# Autodesk Inventor assembly: Montagem eletrolisador sem membrana - sem base
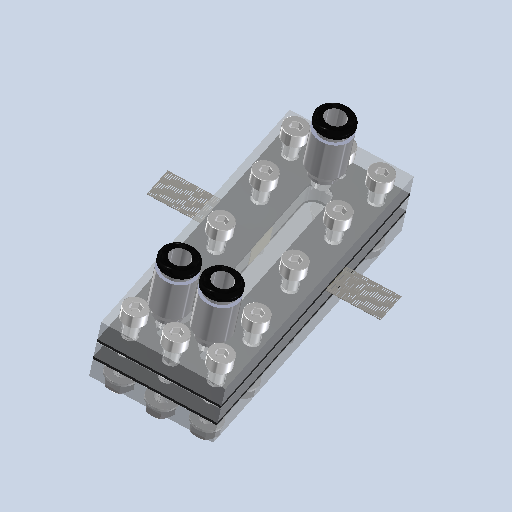
[picture p0: Inventor's stored thumbnail of the model, 512x512]
Saved by Autodesk Inventor 2025 (Build 290162010, 162A)
## iProperties
Created: 2024-12-11
Part Number: Montagem eletrolisador sem membrana - sem base
Document SubType Name: Assembly
Designer: November
Author: November
## Documents named in this file (10)
- G:\Meu Drive\1_Tese 2024\CAD - Eletrolisador\Montagem eletrolisador sem membrana - sem base.iam
- G:\Meu Drive\1_Tese 2024\CAD - Eletrolisador\borracha vedação.ipt
- G:\Meu Drive\1_Tese 2024\CAD - Eletrolisador\acrilico canal.ipt
- G:\Meu Drive\1_Tese 2024\CAD - Eletrolisador\eletrodo - nickel e titanio.ipt
- G:\Meu Drive\1_Tese 2024\CAD - Eletrolisador\acrilico frontal.ipt
- G:\Meu Drive\1_Tese 2024\CAD - Eletrolisador\Screw_DIN_912_M4x25_A2\Screw_DIN_912_M4x25_A2.ipt
- G:\Meu Drive\1_Tese 2024\CAD - Eletrolisador\Engate rápido M5\Engate rápido M5.ipt
- G:\Meu Drive\1_Tese 2024\CAD - Eletrolisador\Arruela m4.ipt
- G:\Meu Drive\1_Tese 2024\CAD - Eletrolisador\PORCA SEXTAVADA M4\PORCA SEXTAVADA M4.ipt
- G:\Meu Drive\1_Tese 2024\CAD - Eletrolisador\acrilico base.ipt
## Components (46 placed, 9 different names)
1. borracha vedação:1 — Alinhado:3, Alinhado:4, Coincidente:6, Coincidente:60
2. acrilico canal:1 — Alinhado:3, Alinhado:4, Coincidente:2, Coincidente:3, Alinhado:5, Coincidente:4, Coincidente:5, Coincidente:6, Alinhado:6, Alinhado:7, Coincidente:61, Coincidente:62
3. eletrodo - nickel e titanio:1 — Coincidente:2, Coincidente:3, Alinhado:5, Coincidente:7
4. eletrodo - nickel e titanio:2 — Coincidente:4, Coincidente:5, Coincidente:7, Coincidente:8
5. borracha vedação:2 — Coincidente:8, Alinhado:6, Alinhado:7, Coincidente:9, Alinhado:8, Alinhado:9, Coincidente:62
6. acrilico frontal:1 — Coincidente:9, Alinhado:8, Alinhado:9, Coincidente:10, Coincidente:11, Coincidente:12, Coincidente:13, Coincidente:14, Coincidente:15, Coincidente:16, Coincidente:17, Coincidente:18, Coincidente:19, Coincidente:20, Coincidente:21, Coincidente:22, Coincidente:23, Coincidente:24, Coincidente:25, Coincidente:26
7. Screw_DIN_912_M4x25_A2:1 — Coincidente:10, Coincidente:11, Alinhado:10, Alinhado:12, Coincidente:27, Coincidente:40
8. Screw_DIN_912_M4x25_A2:2 — Coincidente:12, Alinhado:10, Alinhado:11, Coincidente:38, Coincidente:41
9. Screw_DIN_912_M4x25_A2:3 — Coincidente:13, Alinhado:11, Coincidente:37, Coincidente:42
10. Screw_DIN_912_M4x25_A2:4 — Coincidente:14, Alinhado:13, Coincidente:36, Coincidente:59
11. Screw_DIN_912_M4x25_A2:5 — Coincidente:15, Alinhado:14, Alinhado:20, Coincidente:35, Coincidente:51
12. Screw_DIN_912_M4x25_A2:6 — Coincidente:16, Alinhado:16, Alinhado:20, Coincidente:34, Coincidente:50
13. Screw_DIN_912_M4x25_A2:7 — Coincidente:17, Alinhado:16, Alinhado:17, Coincidente:33, Coincidente:49
14. Screw_DIN_912_M4x25_A2:8 — Coincidente:18, Alinhado:17, Alinhado:18, Coincidente:32, Coincidente:48
15. Screw_DIN_912_M4x25_A2:9 — Coincidente:19, Alinhado:18, Alinhado:19, Coincidente:31, Coincidente:57
16. Screw_DIN_912_M4x25_A2:10 — Coincidente:20, Alinhado:19, Coincidente:30, Coincidente:46
17. Screw_DIN_912_M4x25_A2:11 — Coincidente:21, Alinhado:14, Alinhado:15, Coincidente:29, Coincidente:45
18. Screw_DIN_912_M4x25_A2:12 — Coincidente:22, Alinhado:12, Alinhado:13, Alinhado:15, Coincidente:28, Coincidente:44
19. Engate rápido M5:1 — Coincidente:25, Coincidente:26, Alinhado:21
20. Engate rápido M5:2 — Coincidente:24, Alinhado:21, Alinhado:22
21. Engate rápido M5:3 — Coincidente:23, Alinhado:22
22. Arruela m4:1 — Coincidente:27, Alinhado:23, Alinhado:24, Alinhado:34, Coincidente:52
23. Arruela m4:2 — Coincidente:28, Alinhado:23, Alinhado:33, Alinhado:34, Coincidente:53
24. Arruela m4:3 — Coincidente:29, Alinhado:32, Alinhado:33, Coincidente:54
25. Arruela m4:4 — Coincidente:30, Alinhado:31, Alinhado:32, Coincidente:55
26. Arruela m4:5 — Coincidente:31, Alinhado:30, Alinhado:31, Coincidente:56
27. Arruela m4:6 — Coincidente:32, Alinhado:29, Alinhado:30
28. Arruela m4:7 — Coincidente:33, Alinhado:28, Alinhado:29
29. Arruela m4:8 — Coincidente:34, Alinhado:27, Alinhado:28
30. Arruela m4:9 — Coincidente:35, Alinhado:26, Alinhado:27, Alinhado:35
31. Arruela m4:10 — Coincidente:36, Alinhado:35
32. Arruela m4:11 — Coincidente:37, Alinhado:25, Alinhado:26
33. Arruela m4:12 — Coincidente:38, Alinhado:24, Alinhado:25
34. PORCA SEXTAVADA M4:1 — Coincidente:59, Alinhado:42
35. PORCA SEXTAVADA M4:2 — Coincidente:42, Alinhado:41, Alinhado:42
36. PORCA SEXTAVADA M4:3 — Coincidente:44, Coincidente:53
37. PORCA SEXTAVADA M4:4 — Coincidente:45, Coincidente:54
38. PORCA SEXTAVADA M4:5 — Coincidente:46, Coincidente:55
39. PORCA SEXTAVADA M4:6 — Coincidente:41, Alinhado:40, Alinhado:41
40. PORCA SEXTAVADA M4:7 — Coincidente:49, Alinhado:37, Alinhado:38
41. PORCA SEXTAVADA M4:8 — Coincidente:56, Coincidente:57, Alinhado:36
42. PORCA SEXTAVADA M4:9 — Coincidente:50, Alinhado:38, Alinhado:39
43. PORCA SEXTAVADA M4:10 — Coincidente:48, Alinhado:36, Alinhado:37
44. PORCA SEXTAVADA M4:11 — Coincidente:40, Coincidente:52, Alinhado:40
45. PORCA SEXTAVADA M4:12 — Coincidente:51, Alinhado:39
46. acrilico base:1 — Coincidente:60, Coincidente:61
## Relationships (97: Mate 57, Flush 40)
- Alinhado:3 [Flush]: borracha vedação:1 ↔ acrilico canal:1
- Alinhado:4 [Flush]: borracha vedação:1 ↔ acrilico canal:1
- Coincidente:2 [Mate]: acrilico canal:1 ↔ eletrodo - nickel e titanio:1
- Coincidente:3 [Mate]: acrilico canal:1 ↔ eletrodo - nickel e titanio:1
- Alinhado:5 [Flush] (30 mm): acrilico canal:1 ↔ eletrodo - nickel e titanio:1
- Coincidente:4 [Mate]: acrilico canal:1 ↔ eletrodo - nickel e titanio:2
- Coincidente:5 [Mate]: acrilico canal:1 ↔ eletrodo - nickel e titanio:2
- Coincidente:6 [Mate]: borracha vedação:1 ↔ acrilico canal:1
- Coincidente:7 [Mate]: eletrodo - nickel e titanio:1 ↔ eletrodo - nickel e titanio:2
- Coincidente:8 [Mate]: eletrodo - nickel e titanio:2 ↔ borracha vedação:2
- Alinhado:6 [Flush]: acrilico canal:1 ↔ borracha vedação:2
- Alinhado:7 [Flush]: acrilico canal:1 ↔ borracha vedação:2
- Coincidente:9 [Mate]: borracha vedação:2 ↔ acrilico frontal:1
- Alinhado:8 [Flush]: borracha vedação:2 ↔ acrilico frontal:1
- Alinhado:9 [Flush]: borracha vedação:2 ↔ acrilico frontal:1
- Coincidente:10 [Mate]: acrilico frontal:1 ↔ Screw_DIN_912_M4x25_A2:1
- Coincidente:11 [Mate]: acrilico frontal:1 ↔ Screw_DIN_912_M4x25_A2:1
- Coincidente:12 [Mate]: acrilico frontal:1 ↔ Screw_DIN_912_M4x25_A2:2
- Coincidente:13 [Mate]: acrilico frontal:1 ↔ Screw_DIN_912_M4x25_A2:3
- Coincidente:14 [Mate]: acrilico frontal:1 ↔ Screw_DIN_912_M4x25_A2:4
- Coincidente:15 [Mate]: acrilico frontal:1 ↔ Screw_DIN_912_M4x25_A2:5
- Coincidente:16 [Mate]: acrilico frontal:1 ↔ Screw_DIN_912_M4x25_A2:6
- Coincidente:17 [Mate]: acrilico frontal:1 ↔ Screw_DIN_912_M4x25_A2:7
- Coincidente:18 [Mate]: acrilico frontal:1 ↔ Screw_DIN_912_M4x25_A2:8
- Coincidente:19 [Mate]: acrilico frontal:1 ↔ Screw_DIN_912_M4x25_A2:9
- Coincidente:20 [Mate]: acrilico frontal:1 ↔ Screw_DIN_912_M4x25_A2:10
- Coincidente:21 [Mate]: acrilico frontal:1 ↔ Screw_DIN_912_M4x25_A2:11
- Coincidente:22 [Mate]: acrilico frontal:1 ↔ Screw_DIN_912_M4x25_A2:12
- Alinhado:10 [Flush]: Screw_DIN_912_M4x25_A2:1 ↔ Screw_DIN_912_M4x25_A2:2
- Alinhado:11 [Flush]: Screw_DIN_912_M4x25_A2:2 ↔ Screw_DIN_912_M4x25_A2:3
- Alinhado:12 [Flush]: Screw_DIN_912_M4x25_A2:1 ↔ Screw_DIN_912_M4x25_A2:12
- Alinhado:13 [Flush]: Screw_DIN_912_M4x25_A2:4 ↔ Screw_DIN_912_M4x25_A2:12
- Alinhado:14 [Flush]: Screw_DIN_912_M4x25_A2:5 ↔ Screw_DIN_912_M4x25_A2:11
- Alinhado:15 [Flush]: Screw_DIN_912_M4x25_A2:11 ↔ Screw_DIN_912_M4x25_A2:12
- Alinhado:16 [Flush]: Screw_DIN_912_M4x25_A2:6 ↔ Screw_DIN_912_M4x25_A2:7
- Alinhado:17 [Flush]: Screw_DIN_912_M4x25_A2:7 ↔ Screw_DIN_912_M4x25_A2:8
- Alinhado:18 [Flush]: Screw_DIN_912_M4x25_A2:8 ↔ Screw_DIN_912_M4x25_A2:9
- Alinhado:19 [Flush]: Screw_DIN_912_M4x25_A2:9 ↔ Screw_DIN_912_M4x25_A2:10
- Alinhado:20 [Flush]: Screw_DIN_912_M4x25_A2:5 ↔ Screw_DIN_912_M4x25_A2:6
- Coincidente:23 [Mate]: acrilico frontal:1 ↔ Engate rápido M5:3
- Coincidente:24 [Mate]: acrilico frontal:1 ↔ Engate rápido M5:2
- Coincidente:25 [Mate]: acrilico frontal:1 ↔ Engate rápido M5:1
- Coincidente:26 [Mate] (1 mm): acrilico frontal:1 ↔ Engate rápido M5:1
- Alinhado:21 [Flush]: Engate rápido M5:1 ↔ Engate rápido M5:2
- Alinhado:22 [Flush]: Engate rápido M5:2 ↔ Engate rápido M5:3
- Coincidente:27 [Mate]: Screw_DIN_912_M4x25_A2:1 ↔ Arruela m4:1
- Coincidente:28 [Mate]: Screw_DIN_912_M4x25_A2:12 ↔ Arruela m4:2
- Coincidente:29 [Mate]: Screw_DIN_912_M4x25_A2:11 ↔ Arruela m4:3
- Coincidente:30 [Mate]: Screw_DIN_912_M4x25_A2:10 ↔ Arruela m4:4
- Coincidente:31 [Mate]: Screw_DIN_912_M4x25_A2:9 ↔ Arruela m4:5
- Coincidente:32 [Mate]: Screw_DIN_912_M4x25_A2:8 ↔ Arruela m4:6
- Coincidente:33 [Mate]: Screw_DIN_912_M4x25_A2:7 ↔ Arruela m4:7
- Coincidente:34 [Mate]: Screw_DIN_912_M4x25_A2:6 ↔ Arruela m4:8
- Coincidente:35 [Mate]: Screw_DIN_912_M4x25_A2:5 ↔ Arruela m4:9
- Coincidente:36 [Mate]: Screw_DIN_912_M4x25_A2:4 ↔ Arruela m4:10
- Coincidente:37 [Mate]: Screw_DIN_912_M4x25_A2:3 ↔ Arruela m4:11
- Coincidente:38 [Mate]: Screw_DIN_912_M4x25_A2:2 ↔ Arruela m4:12
- Alinhado:23 [Flush]: Arruela m4:1 ↔ Arruela m4:2
- Alinhado:24 [Flush]: Arruela m4:1 ↔ Arruela m4:12
- Alinhado:25 [Flush]: Arruela m4:11 ↔ Arruela m4:12
- Alinhado:26 [Flush]: Arruela m4:9 ↔ Arruela m4:11
- Alinhado:27 [Flush]: Arruela m4:8 ↔ Arruela m4:9
- Alinhado:28 [Flush]: Arruela m4:7 ↔ Arruela m4:8
- Alinhado:29 [Flush]: Arruela m4:6 ↔ Arruela m4:7
- Alinhado:30 [Flush]: Arruela m4:5 ↔ Arruela m4:6
- Alinhado:31 [Flush]: Arruela m4:4 ↔ Arruela m4:5
- Alinhado:32 [Flush]: Arruela m4:3 ↔ Arruela m4:4
- Alinhado:33 [Flush]: Arruela m4:2 ↔ Arruela m4:3
- Alinhado:34 [Flush]: Arruela m4:1 ↔ Arruela m4:2
- Alinhado:35 [Flush]: Arruela m4:9 ↔ Arruela m4:10
- Coincidente:40 [Mate]: Screw_DIN_912_M4x25_A2:1 ↔ PORCA SEXTAVADA M4:11
- Coincidente:41 [Mate]: Screw_DIN_912_M4x25_A2:2 ↔ PORCA SEXTAVADA M4:6
- Coincidente:42 [Mate]: Screw_DIN_912_M4x25_A2:3 ↔ PORCA SEXTAVADA M4:2
- Coincidente:44 [Mate]: Screw_DIN_912_M4x25_A2:12 ↔ PORCA SEXTAVADA M4:3
- Coincidente:45 [Mate]: Screw_DIN_912_M4x25_A2:11 ↔ PORCA SEXTAVADA M4:4
- Coincidente:46 [Mate]: Screw_DIN_912_M4x25_A2:10 ↔ PORCA SEXTAVADA M4:5
- Coincidente:48 [Mate]: Screw_DIN_912_M4x25_A2:8 ↔ PORCA SEXTAVADA M4:10
- Coincidente:49 [Mate]: Screw_DIN_912_M4x25_A2:7 ↔ PORCA SEXTAVADA M4:7
- Coincidente:50 [Mate]: Screw_DIN_912_M4x25_A2:6 ↔ PORCA SEXTAVADA M4:9
- Coincidente:51 [Mate]: Screw_DIN_912_M4x25_A2:5 ↔ PORCA SEXTAVADA M4:12
- Coincidente:52 [Mate]: Arruela m4:1 ↔ PORCA SEXTAVADA M4:11
- Coincidente:53 [Mate]: Arruela m4:2 ↔ PORCA SEXTAVADA M4:3
- Coincidente:54 [Mate]: Arruela m4:3 ↔ PORCA SEXTAVADA M4:4
- Coincidente:55 [Mate]: Arruela m4:4 ↔ PORCA SEXTAVADA M4:5
- Coincidente:56 [Mate]: Arruela m4:5 ↔ PORCA SEXTAVADA M4:8
- Coincidente:57 [Mate]: Screw_DIN_912_M4x25_A2:9 ↔ PORCA SEXTAVADA M4:8
- Alinhado:36 [Flush]: PORCA SEXTAVADA M4:8 ↔ PORCA SEXTAVADA M4:10
- Alinhado:37 [Flush]: PORCA SEXTAVADA M4:7 ↔ PORCA SEXTAVADA M4:10
- Alinhado:38 [Flush]: PORCA SEXTAVADA M4:7 ↔ PORCA SEXTAVADA M4:9
- Alinhado:39 [Flush]: PORCA SEXTAVADA M4:9 ↔ PORCA SEXTAVADA M4:12
- Alinhado:40 [Flush]: PORCA SEXTAVADA M4:6 ↔ PORCA SEXTAVADA M4:11
- Alinhado:41 [Flush]: PORCA SEXTAVADA M4:2 ↔ PORCA SEXTAVADA M4:6
- Coincidente:59 [Mate]: Screw_DIN_912_M4x25_A2:4 ↔ PORCA SEXTAVADA M4:1
- Alinhado:42 [Flush]: PORCA SEXTAVADA M4:1 ↔ PORCA SEXTAVADA M4:2
- Coincidente:60 [Mate]: borracha vedação:1 ↔ acrilico base:1
- Coincidente:61 [Mate]: acrilico canal:1 ↔ acrilico base:1
- Coincidente:62 [Mate]: acrilico canal:1 ↔ borracha vedação:2
